# Autodesk Inventor assembly: ServoWithShaftAssembly
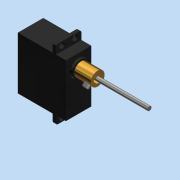
[picture p0: Inventor's stored thumbnail of the model, 180x180]
Saved by Autodesk Inventor 2017 (Build 210142000, 142)
## iProperties
Created: 2016-11-03
Part Number: ServoWithShaftAssembly
Document SubType Name: Assembly
Designer: techn
Author: techn
## Documents named in this file (4)
- E:\OneDrive\Documents\Other Projects\Submarine\CAD\common\3mmShaftToServo\ServoWithShaftAssembly.iam
- E:\OneDrive\Documents\Other Projects\Submarine\CAD\common\HitecServo\HitecServoAssembly.iam
- E:\OneDrive\Documents\Other Projects\Submarine\CAD\common\3mmShaftToServo\.125InchServoDrivenShaft.ipt
- E:\OneDrive\Documents\Other Projects\Submarine\CAD\midships\AftServoSection\ServoShaftCoupler\ServoShaftCouplerAssembly.iam
## Components (3 placed, 3 different names)
1. HitecServoAssembly:1 [sub-assembly] — Mate:1, Mate:2
2. ServoShaftCouplerAssembly:1 [sub-assembly] — Mate:1, Mate:2, Mate:3, Mate:4
3. .125InchServoDrivenShaft:1 — Mate:3, Mate:4
## Relationships (4: Mate 4)
- Mate:1: HitecServoAssembly:1 ↔ ServoShaftCouplerAssembly:1
- Mate:2 (0.254 mm): HitecServoAssembly:1 ↔ ServoShaftCouplerAssembly:1
- Mate:3: ServoShaftCouplerAssembly:1 ↔ .125InchServoDrivenShaft:1
- Mate:4 (0.508 mm): ServoShaftCouplerAssembly:1 ↔ .125InchServoDrivenShaft:1
